# Autodesk Inventor assembly: Full Bot Assembly
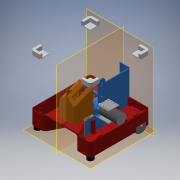
[picture p0: Inventor's stored thumbnail of the model, 180x180]
Saved by Autodesk Inventor 2019 (Build 230136000, 136)
## iProperties
Created: 2019-02-11
Part Number: Full Bot Assembly
Document SubType Name: Assembly
Designer: scigu
Author: scigu
## Documents named in this file (9)
- C:\Users\scigu\Documents\School 18-19\SeCon\Full Bot Assembly.iam
- C:\Users\scigu\Documents\School 18-19\SeCon\Chassis\Chassis--v3-2.ipt
- C:\Users\scigu\Documents\School 18-19\SeCon\Chassis\Caster.ipt
- C:\Users\scigu\Documents\School 18-19\SeCon\Chassis\Small Motor.ipt
- C:\Users\scigu\Documents\School 18-19\SeCon\Chassis\Wheel.ipt
- C:\Users\scigu\Documents\School 18-19\SeCon\Intake\Diverter--v3.ipt
- C:\Users\scigu\Documents\School 18-19\SeCon\Ceiling\Corner Piece.ipt
- C:\Users\scigu\Documents\School 18-19\SeCon\Intake\Wall--v4.ipt
- C:\Users\scigu\Documents\School 18-19\SeCon\Chassis\Big Motor.ipt
## Components (14 placed, 8 different names)
1. Chassis--v3-2:1 — Mate:1, Mate:2, Mate:3, Mate:4, Mate:5, Mate:6, Mate:7, Mate:8, Mate:11, Mate:12, Mate:13, Mate:14, Mate:15, Mate:16, Mate:17, Flush:3, Flush:4, Flush:5, Flush:6, Mate:18, Flush:7, Flush:8, Mate:19, Mate:20, Flush:9, Flush:10, Mate:21, Flush:11, Flush:12, Mate:23, Mate:24
2. Caster:1 — Mate:3, Mate:4, Mate:5
3. Caster:2 — Mate:6, Mate:7, Mate:8, Tangent:1
4. Small Motor:1 — Mate:10, Flush:2, Mate:11, Mate:12, Mate:13
5. Small Motor:2 — Mate:9, Flush:1, Mate:14, Mate:15, Mate:16
6. Wheel:1 — Mate:10, Flush:2
7. Wheel:2 — Mate:9, Flush:1
8. Diverter--v3:1 — Mate:17, Flush:3, Flush:4
9. Corner Piece:1 — Mate:20, Flush:9, Flush:10
10. Corner Piece:2 — Flush:7, Flush:8, Mate:19
11. Corner Piece:3 — Flush:5, Flush:6, Mate:18
12. Corner Piece:4 — Mate:21, Flush:11, Flush:12
13. Wall--v4:1 — Mate:22, Mate:23, Mate:24, Mate:25, Flush:13
14. Big Motor:1 — Mate:25, Flush:13
## Relationships (39: Mate 25, Flush 13, Tangent 1)
- Mate:1: Chassis--v3-2:1
- Mate:2 (111.125 mm): Chassis--v3-2:1
- Mate:3: Chassis--v3-2:1 ↔ Caster:1
- Mate:4: Chassis--v3-2:1 ↔ Caster:1
- Mate:5: Chassis--v3-2:1 ↔ Caster:1
- Mate:6: Chassis--v3-2:1 ↔ Caster:2
- Mate:7: Chassis--v3-2:1 ↔ Caster:2
- Mate:8: Chassis--v3-2:1 ↔ Caster:2
- Tangent:1: Caster:2
- Mate:9: Small Motor:2 ↔ Wheel:2
- Flush:1 (5.08 mm): Small Motor:2 ↔ Wheel:2
- Mate:10: Small Motor:1 ↔ Wheel:1
- Flush:2 (5.08 mm): Small Motor:1 ↔ Wheel:1
- Mate:11: Chassis--v3-2:1 ↔ Small Motor:1
- Mate:12: Chassis--v3-2:1 ↔ Small Motor:1
- Mate:13: Chassis--v3-2:1 ↔ Small Motor:1
- Mate:14: Chassis--v3-2:1 ↔ Small Motor:2
- Mate:15: Chassis--v3-2:1 ↔ Small Motor:2
- Mate:16: Chassis--v3-2:1 ↔ Small Motor:2
- Mate:17: Chassis--v3-2:1 ↔ Diverter--v3:1
- Flush:3: Chassis--v3-2:1 ↔ Diverter--v3:1
- Flush:4: Chassis--v3-2:1 ↔ Diverter--v3:1
- Flush:5: Chassis--v3-2:1 ↔ Corner Piece:3
- Flush:6: Chassis--v3-2:1 ↔ Corner Piece:3
- Mate:18 (177.8 mm): Chassis--v3-2:1 ↔ Corner Piece:3
- Flush:7: Chassis--v3-2:1 ↔ Corner Piece:2
- Flush:8: Chassis--v3-2:1 ↔ Corner Piece:2
- Mate:19 (177.8 mm): Chassis--v3-2:1 ↔ Corner Piece:2
- Mate:20 (177.8 mm): Chassis--v3-2:1 ↔ Corner Piece:1
- Flush:9: Chassis--v3-2:1 ↔ Corner Piece:1
- Flush:10: Chassis--v3-2:1 ↔ Corner Piece:1
- Mate:21 (177.8 mm): Chassis--v3-2:1 ↔ Corner Piece:4
- Flush:11: Chassis--v3-2:1 ↔ Corner Piece:4
- Flush:12: Chassis--v3-2:1 ↔ Corner Piece:4
- Mate:22: Wall--v4:1
- Mate:23: Chassis--v3-2:1 ↔ Wall--v4:1
- Mate:24: Chassis--v3-2:1 ↔ Wall--v4:1
- Mate:25: Wall--v4:1 ↔ Big Motor:1
- Flush:13 (6 mm): Wall--v4:1 ↔ Big Motor:1
